# Autodesk Inventor assembly: ASY BSH 500 cap
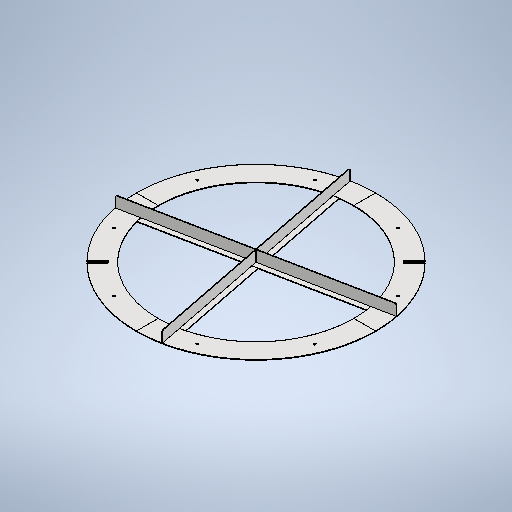
[picture p0: Inventor's stored thumbnail of the model, 512x512]
Saved by Autodesk Inventor 2025 (Build 290162010, 162A)
## iProperties
Created: 2024-09-03
Part Number: ASY BSH 500 cap
Document SubType Name: Assembly
Designer: pokla
Author: pokla
## Documents named in this file (8)
- C:\Users\pokla\Documents\Inventor\BSH_Beshkino_bio_tank\ASY BSH 500 cap.iam
- C:\Users\pokla\Documents\Inventor\BSH_Beshkino_bio_tank\BSH 501 segment.ipt
- C:\Users\pokla\Documents\Inventor\BSH_Beshkino_bio_tank\BSH 502 segment.ipt
- C:\Users\pokla\Documents\Inventor\BSH_Beshkino_bio_tank\BSH 503 inner cross.ipt
- C:\Users\pokla\Documents\Inventor\BSH_Beshkino_bio_tank\BSH DIM 500.1 parameters.ipt
- C:\Users\pokla\Documents\Inventor\BSH_Beshkino_bio_tank\BSH 504 inner cross.ipt
- C:\Users\pokla\Documents\Inventor\BSH_Beshkino_bio_tank\BSH 505 amplifier.ipt
- C:\Users\pokla\Documents\Inventor\BSH_Beshkino_bio_tank\BSH 506 amplifier.ipt
## Components (10 placed, 7 different names)
1. BSH DIM 500.1 parameters:1
2. BSH 501 segment:1 — Rigid:1
3. BSH 501 segment:2 — Rigid:2, Rigid:3
4. BSH 502 segment:1 — Rigid:1, Rigid:2
5. BSH 502 segment:2 — Rigid:3, Rotational:1
6. BSH 503 inner cross:1 — Rotational:1, Rigid:4, Rigid:5, Rigid:7
7. BSH 504 inner cross:1 — Rigid:4
8. BSH 504 inner cross:2 — Rigid:5
9. BSH 505 amplifier:1 — Rigid:7, Rigid:8
10. BSH 506 amplifier:1 — Rigid:8
## Relationships (8: WeldJoint 7, RevoluteJoint 1)
- Rigid:1 [WeldJoint]: BSH 501 segment:1 ↔ BSH 502 segment:1
- Rigid:2 [WeldJoint]: BSH 501 segment:2 ↔ BSH 502 segment:1
- Rigid:3 [WeldJoint]: BSH 501 segment:2 ↔ BSH 502 segment:2
- Rotational:1 [RevoluteJoint]: BSH 502 segment:2 ↔ BSH 503 inner cross:1
- Rigid:4 [WeldJoint]: BSH 503 inner cross:1 ↔ BSH 504 inner cross:1
- Rigid:5 [WeldJoint]: BSH 503 inner cross:1 ↔ BSH 504 inner cross:2
- Rigid:7 [WeldJoint]: BSH 503 inner cross:1 ↔ BSH 505 amplifier:1
- Rigid:8 [WeldJoint] (2 mm): BSH 505 amplifier:1 ↔ BSH 506 amplifier:1
